# Autodesk Inventor assembly: CombinedPiHolder
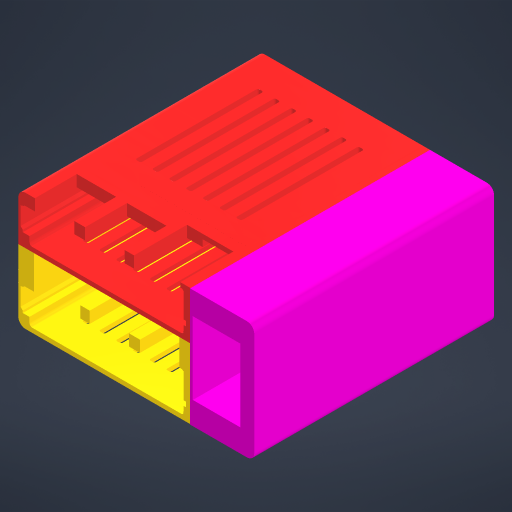
[picture p0: Inventor's stored thumbnail of the model, 512x512]
Saved by Autodesk Inventor 2023 (Build 270158000, 158)
## iProperties
Created: 2023-02-13
Part Number: CombinedPiHolder
Document SubType Name: Assembly
Designer: uzair
Author: uzair
## Documents named in this file (4)
- C:\Users\uzair\Programming\Capstone-MJ02\documentation\3D Models\CombinedPiHolder.iam
- C:\Users\uzair\Programming\Capstone-MJ02\documentation\3D Models\Raspberry_Pi_4_Sleeve_v1-0_MAIN.ipt
- C:\Users\uzair\Programming\Capstone-MJ02\documentation\3D Models\Raspberry_Pi_B+_Sleeve_v2-1_MAIN.ipt
- C:\Users\uzair\Programming\Capstone-MJ02\documentation\3D Models\UE306_Sleeve.ipt
## Components (3 placed, 3 different names)
1. Raspberry_Pi_4_Sleeve_v1-0_MAIN:1 — Mate:1, Mate:2, Mate:3, Mate:4
2. Raspberry_Pi_B+_Sleeve_v2-1_MAIN:1 — Mate:1, Mate:2
3. UE306_Sleeve:1 — Mate:3, Mate:4
## Relationships (4: Mate 4)
- Mate:1: Raspberry_Pi_4_Sleeve_v1-0_MAIN:1 ↔ Raspberry_Pi_B+_Sleeve_v2-1_MAIN:1
- Mate:2: Raspberry_Pi_4_Sleeve_v1-0_MAIN:1 ↔ Raspberry_Pi_B+_Sleeve_v2-1_MAIN:1
- Mate:3: Raspberry_Pi_4_Sleeve_v1-0_MAIN:1 ↔ UE306_Sleeve:1
- Mate:4: Raspberry_Pi_4_Sleeve_v1-0_MAIN:1 ↔ UE306_Sleeve:1
